# Autodesk Inventor assembly: Shooter Curve Assembly
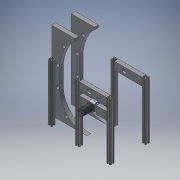
[picture p0: Inventor's stored thumbnail of the model, 180x180]
Saved by Autodesk Inventor 2018 (Build 220112000, 112)
## iProperties
Created: 2020-02-01
Part Number: Shooter Curve Assembly
Document SubType Name: Assembly
Designer: Weeb No1
Author: Weeb No1
## Documents named in this file (6)
- C:\Users\Weeb No1\Documents\GitHub\2020CAD\Gabriel Inventor Files (Shooter, Drivebase)\Shooter Curve Assembly\Main Assembly File\Shooter Curve Assembly.iam
- C:\Users\Weeb No1\Documents\GitHub\2020CAD\Gabriel Inventor Files (Shooter, Drivebase)\Shooter Curve Assembly\Part Files\Shooter Main Curve.ipt
- C:\Users\Weeb No1\Documents\GitHub\2020CAD\Gabriel Inventor Files (Shooter, Drivebase)\Shooter Curve Assembly\Part Files\8020 1010 x 13.ipt
- C:\Users\Weeb No1\Documents\GitHub\2020CAD\Gabriel Inventor Files (Shooter, Drivebase)\Shooter Curve Assembly\Part Files\1x2 5 in Beam Flywheel Mount.ipt
- C:\Users\Weeb No1\Documents\GitHub\2020CAD\Over bumper intake\Parts\VersaPlanetary_v2_Single_Stage_10_1_with_775_Series.iam
- C:\Users\Weeb No1\Documents\GitHub\2020CAD\Gabriel Inventor Files (Shooter, Drivebase)\Shooter Curve Assembly\Part Files\1x2 2 625 in Beam Flywheel Mount.ipt
## Components (15 placed, 5 different names)
1. Shooter Main Curve:1 — Flush:1, Mate:1, Mate:2, Flush:2, Flush:3, Flush:18, Flush:20, Flush:30, Mate:15, Flush:32, Flush:33
2. 8020 1010 x 13:1 — Flush:1, Mate:1, Flush:5, Flush:6, Mate:7, Flush:11, Flush:14, Flush:18, Flush:23, Flush:24, Mate:17, Flush:35
3. 8020 1010 x 13:2 — Flush:4, Mate:3, Flush:7, Mate:9, Flush:15, Flush:19, Flush:22, Flush:25
4. Shooter Main Curve:2 — Mate:2, Flush:2, Flush:3, Flush:4, Mate:3, Flush:19, Flush:21, Mate:14, Flush:31
5. 8020 1010 x 13:3 — Flush:5, Flush:6, Flush:10, Flush:12, Flush:13, Flush:20, Mate:11, Flush:23, Mate:12, Flush:28, Flush:29, Mate:16, Flush:34
6. 8020 1010 x 13:4 — Flush:7, Flush:10, Flush:17, Flush:21, Mate:10, Flush:22, Mate:13, Flush:26, Flush:27
7. 1x2 5 in Beam Flywheel Mount:1 — Mate:9, Flush:15, Flush:17, Mate:10, Flush:25
8. 1x2 5 in Beam Flywheel Mount:2 — Mate:7, Flush:11, Flush:12, Flush:13, Flush:14, Mate:11, Flush:24
9. 8020 1010 x 13:5 — Mate:13, Flush:26, Flush:27
10. 8020 1010 x 13:6 — Mate:12, Flush:28, Flush:29
11. 8020 1010 x 13:7 — Flush:30, Mate:14, Flush:31
12. 8020 1010 x 13:8 — Mate:15, Flush:32, Flush:33
13. VersaPlanetary_v2_Single_Stage_10_1_with_775_Series:1 [sub-assembly] — Mate:18, Mate:19
14. 1x2 2 625 in Beam Flywheel Mount:1 — Mate:17, Flush:35, Flush:36, Mate:19
15. 1x2 2 625 in Beam Flywheel Mount:2 — Mate:16, Flush:34, Flush:36, Mate:18
## Relationships (48: Flush 33, Mate 15)
- Flush:1 (203.2 mm): Shooter Main Curve:1 ↔ 8020 1010 x 13:1
- Mate:1 (25.4 mm): Shooter Main Curve:1 ↔ 8020 1010 x 13:1
- Mate:2 (101.6 mm): Shooter Main Curve:1 ↔ Shooter Main Curve:2
- Flush:2: Shooter Main Curve:1 ↔ Shooter Main Curve:2
- Flush:3: Shooter Main Curve:1 ↔ Shooter Main Curve:2
- Flush:4 (203.2 mm): 8020 1010 x 13:2 ↔ Shooter Main Curve:2
- Mate:3 (25.4 mm): 8020 1010 x 13:2 ↔ Shooter Main Curve:2
- Flush:5: 8020 1010 x 13:1 ↔ 8020 1010 x 13:3
- Flush:6: 8020 1010 x 13:1 ↔ 8020 1010 x 13:3
- Flush:7: 8020 1010 x 13:2 ↔ 8020 1010 x 13:4
- Flush:10: 8020 1010 x 13:3 ↔ 8020 1010 x 13:4
- Mate:7: 8020 1010 x 13:1 ↔ 1x2 5 in Beam Flywheel Mount:2
- Flush:11: 8020 1010 x 13:1 ↔ 1x2 5 in Beam Flywheel Mount:2
- Flush:12: 8020 1010 x 13:3 ↔ 1x2 5 in Beam Flywheel Mount:2
- Flush:13: 8020 1010 x 13:3 ↔ 1x2 5 in Beam Flywheel Mount:2
- Flush:14: 8020 1010 x 13:1 ↔ 1x2 5 in Beam Flywheel Mount:2
- Mate:9: 8020 1010 x 13:2 ↔ 1x2 5 in Beam Flywheel Mount:1
- Flush:15: 8020 1010 x 13:2 ↔ 1x2 5 in Beam Flywheel Mount:1
- Flush:17: 8020 1010 x 13:4 ↔ 1x2 5 in Beam Flywheel Mount:1
- Flush:18 (-37.846 mm): Shooter Main Curve:1 ↔ 8020 1010 x 13:1
- Flush:19 (-37.846 mm): 8020 1010 x 13:2 ↔ Shooter Main Curve:2
- Flush:20 (-37.846 mm): Shooter Main Curve:1 ↔ 8020 1010 x 13:3
- Flush:21 (-37.846 mm): Shooter Main Curve:2 ↔ 8020 1010 x 13:4
- Mate:10: 8020 1010 x 13:4 ↔ 1x2 5 in Beam Flywheel Mount:1
- Mate:11: 8020 1010 x 13:3 ↔ 1x2 5 in Beam Flywheel Mount:2
- Flush:22: 8020 1010 x 13:2 ↔ 8020 1010 x 13:4
- Flush:23: 8020 1010 x 13:1 ↔ 8020 1010 x 13:3
- Flush:24: 8020 1010 x 13:1 ↔ 1x2 5 in Beam Flywheel Mount:2
- Flush:25: 8020 1010 x 13:2 ↔ 1x2 5 in Beam Flywheel Mount:1
- Mate:12 (127 mm): 8020 1010 x 13:3 ↔ 8020 1010 x 13:6
- Mate:13 (127 mm): 8020 1010 x 13:4 ↔ 8020 1010 x 13:5
- Flush:26: 8020 1010 x 13:4 ↔ 8020 1010 x 13:5
- Flush:27: 8020 1010 x 13:4 ↔ 8020 1010 x 13:5
- Flush:28: 8020 1010 x 13:3 ↔ 8020 1010 x 13:6
- Flush:29: 8020 1010 x 13:3 ↔ 8020 1010 x 13:6
- Flush:30: Shooter Main Curve:1 ↔ 8020 1010 x 13:7
- Mate:14: Shooter Main Curve:2 ↔ 8020 1010 x 13:7
- Flush:31 (-37.846 mm): Shooter Main Curve:2 ↔ 8020 1010 x 13:7
- Mate:15: Shooter Main Curve:1 ↔ 8020 1010 x 13:8
- Flush:32: Shooter Main Curve:1 ↔ 8020 1010 x 13:8
- Flush:33 (-37.846 mm): Shooter Main Curve:1 ↔ 8020 1010 x 13:8
- Mate:16: 8020 1010 x 13:3 ↔ 1x2 2 625 in Beam Flywheel Mount:2
- Flush:34: 8020 1010 x 13:3 ↔ 1x2 2 625 in Beam Flywheel Mount:2
- Mate:17: 8020 1010 x 13:1 ↔ 1x2 2 625 in Beam Flywheel Mount:1
- Flush:35: 8020 1010 x 13:1 ↔ 1x2 2 625 in Beam Flywheel Mount:1
- Flush:36: 1x2 2 625 in Beam Flywheel Mount:1 ↔ 1x2 2 625 in Beam Flywheel Mount:2
- Mate:18: VersaPlanetary_v2_Single_Stage_10_1_with_775_Series:1 ↔ 1x2 2 625 in Beam Flywheel Mount:2
- Mate:19: VersaPlanetary_v2_Single_Stage_10_1_with_775_Series:1 ↔ 1x2 2 625 in Beam Flywheel Mount:1
